# Autodesk Inventor assembly: Newone
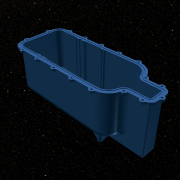
[picture p0: Inventor's stored thumbnail of the model, 180x180]
Saved by Autodesk Inventor 2012 (Build 160160000, 160)
## iProperties
Created: 2012-10-11
Part Number: Newone
Document SubType Name: Assembly
Designer: SONY
Author: SONY
## Documents named in this file (9)
- C:\Users\SONY\Desktop\XRAY\newxrt2\New-XRT.iam
- C:\Users\SONY\Desktop\XRAY\newxrt2\TSC-102-57-25.ipt
- C:\Users\SONY\Desktop\XRAY\newxrt2\Primary.ipt
- C:\Users\SONY\Desktop\XRAY\newxrt2\HV-Inner.ipt
- C:\Users\SONY\Desktop\XRAY\newxrt2\HV-Outer.ipt
- C:\Users\SONY\Desktop\XRAY\newxrt2\oilcase-1.ipt
- C:\Users\SONY\Desktop\XRAY\newxrt2\Divider.ipt
- C:\Users\SONY\Desktop\XRAY\newxrt2\oilcaselid.ipt
- C:\Users\SONY\Desktop\XRAY\newxrt2\New-XRT\Design Accelerator\Bolted Connection1.iam
## Components (10 placed, 8 different names)
1. TSC-102-57-25:1 — Mate:1, Flush:1, Flush:2, Flush:6
2. TSC-102-57-25:2 — Mate:1, Flush:1, Flush:2, Flush:3, Flush:4
3. Primary_Bobbin — Flush:3
4. HV_Bobbin — Flush:4, Flush:5
5. HV-Outer:1 — Flush:5
6. oilcase-1:1 — Flush:6, Flush:7, Mate:7, Mate:8, Mate:9, Mate:11, Mate:12, Flush:8, Flush:9
7. Divider:1 — Flush:7
8. Bolted Connection:1 [sub-assembly] — Mate:11
9. Divider:2 — Mate:7, Mate:8, Mate:9
10. oilcaselid:1 — Mate:12, Flush:8, Flush:9
## Relationships (15: Flush 9, Mate 6)
- Mate:1: TSC-102-57-25:1 ↔ TSC-102-57-25:2
- Flush:1: TSC-102-57-25:1 ↔ TSC-102-57-25:2
- Flush:2: TSC-102-57-25:1 ↔ TSC-102-57-25:2
- Flush:3: TSC-102-57-25:2 ↔ Primary_Bobbin
- Flush:4: TSC-102-57-25:2 ↔ HV_Bobbin
- Flush:5: HV_Bobbin ↔ HV-Outer:1
- Flush:6: TSC-102-57-25:1 ↔ oilcase-1:1
- Flush:7: oilcase-1:1 ↔ Divider:1
- Mate:7: oilcase-1:1 ↔ Divider:2
- Mate:8: oilcase-1:1 ↔ Divider:2
- Mate:9: oilcase-1:1 ↔ Divider:2
- Mate:11: oilcase-1:1 ↔ Bolted Connection:1
- Mate:12: oilcase-1:1 ↔ oilcaselid:1
- Flush:8: oilcase-1:1 ↔ oilcaselid:1
- Flush:9: oilcase-1:1 ↔ oilcaselid:1
